# Autodesk Inventor assembly: Roller Carouel Assembly
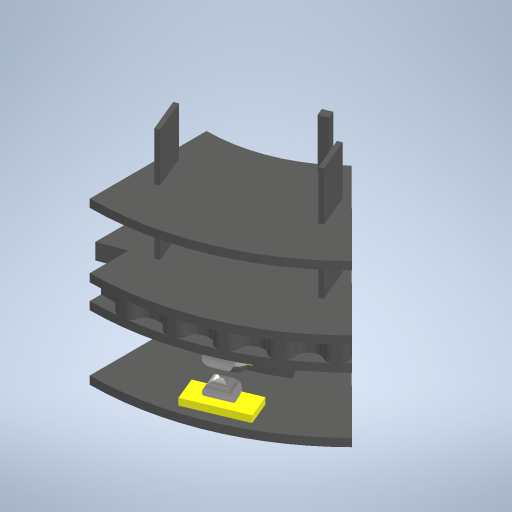
[picture p0: Inventor's stored thumbnail of the model, 512x512]
Saved by Autodesk Inventor 2023 (Build 270158000, 158)
## iProperties
Created: 2022-11-09
Part Number: Roller Carouel Assembly
Document SubType Name: Assembly
Designer: cheng
Mass: 2238.02 g
Surface Area: 4892.44 cm^2
Volume: 2375.07 cm^3
Density: 0.942297 g/cm^3
Author: cheng
## Documents named in this file (6)
- C:\Users\mihal\Desktop\4th Year Project\BHSS DESIGN\Sixth Assembly\Roller Carouel Assembly.iam
- C:\Users\mihal\Desktop\4th Year Project\BHSS DESIGN\Sixth Assembly\Roller Carousel Part.ipt
- C:\Users\mihal\Desktop\4th Year Project\BHSS DESIGN\Sixth Assembly\6002-z-bnl v1.ipt
- C:\Users\mihal\Desktop\4th Year Project\BHSS DESIGN\Sixth Assembly\Carousel Container Plate.ipt
- C:\Users\mihal\Desktop\4th Year Project\BHSS DESIGN\Sixth Assembly\Roller Carousel Gear.ipt
- C:\Users\mihal\Desktop\4th Year Project\BHSS DESIGN\Sixth Assembly\Ball Transfer Unit Assembly.iam
## Components (9 placed, 5 different names)
1. Roller Carousel Part:1 — Mate:7, Mate:8, Mate:13, Mate:14, Mate:15, Mate:16, Mate:17, Mate:18, Mate:19, Mate:20, Mate:21, Mate:22, Mate:23, Mate:24, Mate:25, Mate:26
2. Carousel Container Plate:1 — Mate:10, Mate:11, Mate:12
3. Roller Carousel Gear:1 — Mate:7, Mate:8, Mate:10, Mate:11, Mate:12
4. Ball Transfer Unit Assembly:1 [sub-assembly] — Mate:19, Mate:20
5. Ball Transfer Unit Assembly:2 [sub-assembly] — Mate:17, Mate:18
6. 6002-z-bnl v1:1 — Mate:15, Mate:16
7. 6002-z-bnl v1:2 — Mate:13, Mate:14
8. Ball Transfer Unit Assembly:3 [sub-assembly] — Mate:21, Mate:23, Mate:24
9. Ball Transfer Unit Assembly:4 [sub-assembly] — Mate:22, Mate:25, Mate:26
## Relationships (19: Mate 19)
- Mate:7: Roller Carousel Part:1 ↔ Roller Carousel Gear:1
- Mate:8: Roller Carousel Part:1 ↔ Roller Carousel Gear:1
- Mate:10: Carousel Container Plate:1 ↔ Roller Carousel Gear:1
- Mate:11: Carousel Container Plate:1 ↔ Roller Carousel Gear:1
- Mate:12: Carousel Container Plate:1 ↔ Roller Carousel Gear:1
- Mate:13: Roller Carousel Part:1 ↔ 6002-z-bnl v1:2
- Mate:14: Roller Carousel Part:1 ↔ 6002-z-bnl v1:2
- Mate:15: Roller Carousel Part:1 ↔ 6002-z-bnl v1:1
- Mate:16: Roller Carousel Part:1 ↔ 6002-z-bnl v1:1
- Mate:17: Roller Carousel Part:1 ↔ Ball Transfer Unit Assembly:2
- Mate:18: Roller Carousel Part:1 ↔ Ball Transfer Unit Assembly:2
- Mate:19: Roller Carousel Part:1 ↔ Ball Transfer Unit Assembly:1
- Mate:20: Roller Carousel Part:1 ↔ Ball Transfer Unit Assembly:1
- Mate:21: Roller Carousel Part:1 ↔ Ball Transfer Unit Assembly:3
- Mate:22: Roller Carousel Part:1 ↔ Ball Transfer Unit Assembly:4
- Mate:23: Roller Carousel Part:1 ↔ Ball Transfer Unit Assembly:3
- Mate:24: Roller Carousel Part:1 ↔ Ball Transfer Unit Assembly:3
- Mate:25: Roller Carousel Part:1 ↔ Ball Transfer Unit Assembly:4
- Mate:26: Roller Carousel Part:1 ↔ Ball Transfer Unit Assembly:4
